# Autodesk Inventor assembly: 12mm Incremental Encoder - BOURNS PEC11S
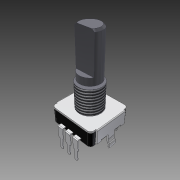
[picture p0: Inventor's stored thumbnail of the model, 180x180]
Saved by Autodesk Inventor 2014 (Build 180170000, 170)
## iProperties
Created: 2011-11-07
Part Number: 12mm Incremental Encoder - BOURNS PEC11S
Document SubType Name: Assembly
Designer: sdarley
Author: sdarley
## Documents named in this file (9)
- C:\Users\buben\Documents\GitHub\bacon\inventor files\3rd party components\rotary_encoder\12mm Incremental Encoder - BOURNS PEC11S.iam
- C:\Users\buben\Documents\GitHub\bacon\inventor files\3rd party components\rotary_encoder\12mm Incremental Encoder Base.ipt
- C:\Users\buben\Documents\GitHub\bacon\inventor files\3rd party components\rotary_encoder\12mm Incremental Encoder Pin.ipt
- C:\Users\buben\Documents\GitHub\bacon\inventor files\3rd party components\rotary_encoder\12mm Incremental Encoder Anti-Rotation Plate.ipt
- C:\Users\buben\Documents\GitHub\bacon\inventor files\3rd party components\rotary_encoder\12mm Incremental Encoder Threaded Tube.ipt
- C:\Users\buben\Documents\GitHub\bacon\inventor files\3rd party components\rotary_encoder\12mm Incremental Encoder Washer.ipt
- C:\Users\buben\Documents\GitHub\bacon\inventor files\3rd party components\rotary_encoder\M7x0.75 Hex Nut.ipt
- C:\Users\buben\Documents\GitHub\bacon\inventor files\3rd party components\rotary_encoder\12mm Incremental Encoder Shaft.ipt
- C:\Users\buben\Documents\GitHub\bacon\inventor files\3rd party components\rotary_encoder\12mm Incremental Encoder Cap.ipt
## Components (12 placed, 8 different names)
1. 12mm Incremental Encoder Base:1 — Mate:1, Mate:2, Mate:3, Mate:4, Mate:5, Mate:6, Mate:7, Mate:8, Flush:1, Flush:2, Flush:3, Flush:4, Flush:5, Flush:6, Flush:7, Flush:8
2. 12mm Incremental Encoder Pin:1 — Mate:3, Mate:6, Flush:2
3. 12mm Incremental Encoder Pin:2 — Mate:4, Flush:4, Flush:6
4. 12mm Incremental Encoder Pin:3 — Mate:5, Flush:5, Flush:7
5. 12mm Incremental Encoder Pin:4 — Mate:1, Mate:8, Flush:1
6. 12mm Incremental Encoder Pin:5 — Mate:2, Mate:7, Flush:3
7. 12mm Incremental Encoder Anti-Rotation Plate:1 — Flush:8, Flush:9, Flush:10
8. 12mm Incremental Encoder Threaded Tube:1 — Flush:9, Mate:9, Flush:11
9. 12mm Incremental Encoder Washer:1 — Flush:10, Mate:10
10. M7x0.75 Hex Nut:1 — Mate:9, Mate:10
11. 12mm Incremental Encoder Shaft:1 — Flush:11, Flush:12
12. 12mm Incremental Encoder Cap:1 — Flush:12
## Relationships (22: Flush 12, Mate 10)
- Mate:1: 12mm Incremental Encoder Base:1 ↔ 12mm Incremental Encoder Pin:4
- Mate:2: 12mm Incremental Encoder Base:1 ↔ 12mm Incremental Encoder Pin:5
- Mate:3: 12mm Incremental Encoder Base:1 ↔ 12mm Incremental Encoder Pin:1
- Mate:4: 12mm Incremental Encoder Base:1 ↔ 12mm Incremental Encoder Pin:2
- Mate:5: 12mm Incremental Encoder Base:1 ↔ 12mm Incremental Encoder Pin:3
- Mate:6: 12mm Incremental Encoder Base:1 ↔ 12mm Incremental Encoder Pin:1
- Mate:7 (2.5 mm): 12mm Incremental Encoder Base:1 ↔ 12mm Incremental Encoder Pin:5
- Mate:8 (-2.5 mm): 12mm Incremental Encoder Base:1 ↔ 12mm Incremental Encoder Pin:4
- Flush:1 (-3 mm): 12mm Incremental Encoder Base:1 ↔ 12mm Incremental Encoder Pin:4
- Flush:2 (-3 mm): 12mm Incremental Encoder Base:1 ↔ 12mm Incremental Encoder Pin:1
- Flush:3 (-3 mm): 12mm Incremental Encoder Base:1 ↔ 12mm Incremental Encoder Pin:5
- Flush:4 (2.5 mm): 12mm Incremental Encoder Base:1 ↔ 12mm Incremental Encoder Pin:2
- Flush:5 (2.5 mm): 12mm Incremental Encoder Base:1 ↔ 12mm Incremental Encoder Pin:3
- Flush:6 (-3 mm): 12mm Incremental Encoder Base:1 ↔ 12mm Incremental Encoder Pin:2
- Flush:7 (-3 mm): 12mm Incremental Encoder Base:1 ↔ 12mm Incremental Encoder Pin:3
- Flush:8: 12mm Incremental Encoder Base:1 ↔ 12mm Incremental Encoder Anti-Rotation Plate:1
- Flush:9: 12mm Incremental Encoder Anti-Rotation Plate:1 ↔ 12mm Incremental Encoder Threaded Tube:1
- Flush:10 (2 mm): 12mm Incremental Encoder Anti-Rotation Plate:1 ↔ 12mm Incremental Encoder Washer:1
- Mate:9: 12mm Incremental Encoder Threaded Tube:1 ↔ M7x0.75 Hex Nut:1
- Mate:10: 12mm Incremental Encoder Washer:1 ↔ M7x0.75 Hex Nut:1
- Flush:11: 12mm Incremental Encoder Threaded Tube:1 ↔ 12mm Incremental Encoder Shaft:1
- Flush:12 (1 mm): 12mm Incremental Encoder Shaft:1 ↔ 12mm Incremental Encoder Cap:1
